# Autodesk Inventor assembly: левый привод_MIR1
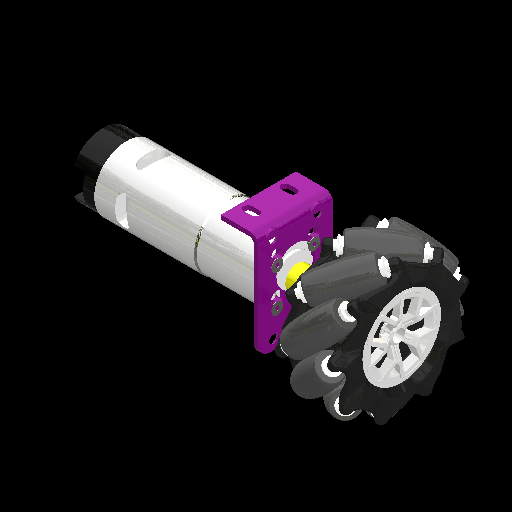
[picture p0: Inventor's stored thumbnail of the model, 512x512]
Saved by Autodesk Inventor 2025 (Build 290162000, 162)
## iProperties
Created: 2025-02-16
Part Number: левый привод_MIR1
Document SubType Name: Assembly
Designer: volko
Author: volko
## Documents named in this file (8)
- C:\Users\volko\Desktop\диплом\Модели\детали\левый привод_MIR1.iam
- C:\Users\volko\Desktop\диплом\Модели\детали\CHP-42GP-775 ABHL_MIR_MIR1.ipt
- C:\Users\volko\Desktop\диплом\Модели\детали\кронштейн_MIR_MIR1.ipt
- C:\Users\volko\Desktop\диплом\Модели\детали\переходная втулка_MIR_MIR1.ipt
- C:\Users\volko\Desktop\диплом\Модели\Mecanum wheel - left\Mecanum wheel - left_MIR1.iam
- C:\Users\volko\Desktop\диплом\Модели\детали\стандартные изделия\ru-RU\DIN 7991(2)\DIN 7991 - M4x8.ipt
- C:\Users\volko\Desktop\диплом\Модели\детали\стандартные изделия\ru-RU\ISO 7380-1\ISO 7380-1 - M4 x 25.ipt
- C:\Users\volko\Desktop\диплом\Модели\детали\стандартные изделия\ru-RU\DIN 913\DIN 913 - M3 x 4.ipt
## Components (10 placed, 7 different names)
1. CHP-42GP-775 ABHL_MIR_MIR1:1 — Заподлицо:1, Совмещение:2, Совмещение:1, Совмещение:11, Совмещение:7, Совмещение:5, Совмещение:4, Совмещение:3, Совмещение:19
2. кронштейн_MIR_MIR1:1 — Совмещение:11, Совмещение:7, Совмещение:5, Совмещение:11, Совмещение:12, Совмещение:13, Совмещение:14
3. переходная втулка_MIR_MIR1:1 — Совмещение:4, Совмещение:3, Совмещение:10, Совмещение:9, Совмещение:8, Совмещение:16, Совмещение:18
4. Mecanum wheel - left_MIR1:1 [sub-assembly] — Совмещение:10, Совмещение:9, Совмещение:8, Совмещение:15, Совмещение:17
5. DIN 913 M3 x 4:1 — Совмещение:16, Совмещение:19
6. ISO 7380-1 M4 x 25:1 — Совмещение:15, Совмещение:17
7. DIN 7991 M4x8:4 — Совмещение:14
8. DIN 7991 M4x8:3 — Совмещение:13
9. DIN 7991 M4x8:2 — Совмещение:12
10. DIN 7991 M4x8:1 — Совмещение:11
## Relationships (20: Mate 19, Flush 1)
- Заподлицо:1 [Flush]: CHP-42GP-775 ABHL_MIR_MIR1:1
- Совмещение:2 [Mate]: CHP-42GP-775 ABHL_MIR_MIR1:1
- Совмещение:1 [Mate]: CHP-42GP-775 ABHL_MIR_MIR1:1
- Совмещение:11 [Mate]: CHP-42GP-775 ABHL_MIR_MIR1:1 ↔ кронштейн_MIR_MIR1:1
- Совмещение:7 [Mate]: CHP-42GP-775 ABHL_MIR_MIR1:1 ↔ кронштейн_MIR_MIR1:1
- Совмещение:5 [Mate]: CHP-42GP-775 ABHL_MIR_MIR1:1 ↔ кронштейн_MIR_MIR1:1
- Совмещение:4 [Mate]: CHP-42GP-775 ABHL_MIR_MIR1:1 ↔ переходная втулка_MIR_MIR1:1
- Совмещение:3 [Mate]: CHP-42GP-775 ABHL_MIR_MIR1:1 ↔ переходная втулка_MIR_MIR1:1
- Совмещение:10 [Mate]: переходная втулка_MIR_MIR1:1 ↔ Mecanum wheel - left_MIR1:1
- Совмещение:9 [Mate]: переходная втулка_MIR_MIR1:1 ↔ Mecanum wheel - left_MIR1:1
- Совмещение:8 [Mate]: переходная втулка_MIR_MIR1:1 ↔ Mecanum wheel - left_MIR1:1
- Совмещение:11 [Mate]: кронштейн_MIR_MIR1:1 ↔ DIN 7991 M4x8:1
- Совмещение:12 [Mate]: кронштейн_MIR_MIR1:1 ↔ DIN 7991 M4x8:2
- Совмещение:13 [Mate]: кронштейн_MIR_MIR1:1 ↔ DIN 7991 M4x8:3
- Совмещение:14 [Mate]: кронштейн_MIR_MIR1:1 ↔ DIN 7991 M4x8:4
- Совмещение:15 [Mate]: Mecanum wheel - left_MIR1:1 ↔ ISO 7380-1 M4 x 25:1
- Совмещение:16 [Mate]: переходная втулка_MIR_MIR1:1 ↔ DIN 913 M3 x 4:1
- Совмещение:17 [Mate]: Mecanum wheel - left_MIR1:1 ↔ ISO 7380-1 M4 x 25:1
- Совмещение:18 [Mate]: переходная втулка_MIR_MIR1:1
- Совмещение:19 [Mate]: CHP-42GP-775 ABHL_MIR_MIR1:1 ↔ DIN 913 M3 x 4:1
